# Autodesk Inventor assembly: robot
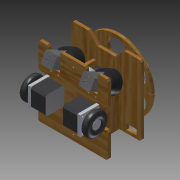
[picture p0: Inventor's stored thumbnail of the model, 180x180]
Saved by Autodesk Inventor 2013 (Build 170138000, 138)
## iProperties
Created: 2013-07-24
Part Number: robot
Document SubType Name: Assembly
Designer: dkboone
Author: dkboone
## Documents named in this file (11)
- J:\groups\theresistors\Inventor\robot.iam
- J:\groups\theresistors\Inventor\base.ipt
- J:\groups\theresistors\Inventor\wheel_assembly.iam
- J:\groups\theresistors\Inventor\carousel_base.ipt
- J:\groups\theresistors\Inventor\carousel.ipt
- J:\groups\theresistors\Inventor\ping_pong_ball.ipt
- J:\groups\theresistors\Inventor\launcher_assembly.iam
- J:\groups\theresistors\Inventor\stepper_short.ipt
- J:\groups\theresistors\Inventor\chute_wall.ipt
- J:\groups\theresistors\Inventor\chute_back.ipt
- J:\groups\theresistors\Inventor\carousel_hub.ipt
## Components (14 placed, 10 different names)
1. base:1 — Mate:1, Mate:2, Mate:3, Mate:4, Mate:5, Mate:6, Angle:4, Angle:5, Mate:13, Mate:14, Mate:15, Mate:16, Flush:8, Flush:9, Mate:17, Flush:10, Flush:12, Flush:13
2. wheel_assembly:1 [sub-assembly] — Mate:1, Mate:2, Mate:3
3. wheel_assembly:2 [sub-assembly] — Mate:4, Mate:5, Mate:6
4. carousel_base:1 — Mate:8, Mate:21, Flush:12, Flush:13
5. carousel:1 — Mate:8, Mate:10, Mate:22
6. ping_pong_ball:1 — Mate:10
7. ping_pong_ball:2
8. stepper_short:1 — Mate:23
9. launcher_assembly:1 [sub-assembly] — Angle:4, Mate:13, Flush:6, Flush:7
10. launcher_assembly:2 [sub-assembly] — Angle:5, Flush:6, Mate:14, Flush:7, Mate:15
11. chute_wall:1 — Mate:16, Flush:8, Flush:9, Mate:18, Mate:19, Flush:11, Mate:21
12. chute_wall:2 — Mate:17, Flush:10, Mate:18, Mate:20
13. chute_back:1 — Mate:19, Mate:20, Flush:11
14. carousel_hub:1 — Mate:22, Mate:23
## Relationships (29: Mate 19, Flush 8, Angle 2)
- Mate:1: base:1 ↔ wheel_assembly:1
- Mate:2: base:1 ↔ wheel_assembly:1
- Mate:3: base:1 ↔ wheel_assembly:1
- Mate:4: base:1 ↔ wheel_assembly:2
- Mate:5: base:1 ↔ wheel_assembly:2
- Mate:6: base:1 ↔ wheel_assembly:2
- Mate:8 (16.764 mm): carousel_base:1 ↔ carousel:1
- Mate:10: carousel:1 ↔ ping_pong_ball:1
- Angle:4 (-118 deg): base:1 ↔ launcher_assembly:1
- Angle:5 (-118 deg): base:1 ↔ launcher_assembly:2
- Mate:13: base:1 ↔ launcher_assembly:1
- Flush:6: launcher_assembly:1 ↔ launcher_assembly:2
- Mate:14: base:1 ↔ launcher_assembly:2
- Flush:7: launcher_assembly:1 ↔ launcher_assembly:2
- Mate:15: base:1 ↔ launcher_assembly:2
- Mate:16: base:1 ↔ chute_wall:1
- Flush:8: base:1 ↔ chute_wall:1
- Flush:9 (-47.625 mm): base:1 ↔ chute_wall:1
- Mate:17: base:1 ↔ chute_wall:2
- Flush:10: base:1 ↔ chute_wall:2
- Mate:18 (44.45 mm): chute_wall:1 ↔ chute_wall:2
- Mate:19: chute_wall:1 ↔ chute_back:1
- Mate:20: chute_wall:2 ↔ chute_back:1
- Flush:11: chute_wall:1 ↔ chute_back:1
- Mate:21: carousel_base:1 ↔ chute_wall:1
- Flush:12: base:1 ↔ carousel_base:1
- Flush:13: base:1 ↔ carousel_base:1
- Mate:22: carousel:1 ↔ carousel_hub:1
- Mate:23: stepper_short:1 ↔ carousel_hub:1
